# Autodesk Inventor assembly: A2017_T5_08
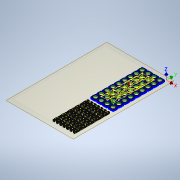
[picture p0: Inventor's stored thumbnail of the model, 180x180]
Saved by Autodesk Inventor 2022 (Build 260153000, 153)
## iProperties
Created: 2022-09-28
Part Number: A2017_T5_08
Document SubType Name: Assembly
Designer: Masato
Author: Masato
## Documents named in this file (6)
- C:\Users\ヨコオリク\Documents\CITBrains\SUSTAINA-OP\Cam\A2017_T5\A2017_T5_08.iam
- C:\Users\ヨコオリク\Documents\CITBrains\SUSTAINA-OP\Cam\DisposableBoard.ipt
- C:\Users\ヨコオリク\Documents\CITBrains\SUSTAINA-OP\LowerBody\Knee\Knee_clamp.ipt
- C:\Users\ヨコオリク\Documents\CITBrains\SUSTAINA-OP\UpperBody\Trunk\CrossRollerBearing\Inner_support_stand.ipt
- C:\Users\ヨコオリク\Documents\CITBrains\SUSTAINA-OP\UpperBody\Trunk\CrossRollerBearing\Outer_support_stand.ipt
- C:\Users\ヨコオリク\Documents\CITBrains\SUSTAINA-OP\LowerBody\Foot\Foot_root_block.ipt
## Components (103 placed, 5 different names)
1. DisposableBoard:1 — フラッシュ:1, フラッシュ:2, フラッシュ:3, フラッシュ:4, 正接:1, 正接:2, 正接:7, 正接:12, 正接:13, フラッシュ:5, フラッシュ:6, 正接:15, 正接:16
2. Inner_support_stand:1 — メイト:2, 挿入:1, 角度:2
3. Outer_support_stand:1 — メイト:1, 角度:1, 正接:1, 正接:2, 挿入:1
4. Inner_support_stand:2
5. Outer_support_stand:2
6. Inner_support_stand:3
7. Outer_support_stand:3
8. Inner_support_stand:4
9. Outer_support_stand:4
10. Inner_support_stand:5
11. Outer_support_stand:5
12. Inner_support_stand:6
13. Outer_support_stand:6
14. Inner_support_stand:7
15. Outer_support_stand:7
16. Inner_support_stand:8
17. Outer_support_stand:8
18. Inner_support_stand:9
19. Outer_support_stand:9
20. Inner_support_stand:10
21. Outer_support_stand:10
22. Knee_clamp:1 — メイト:4, メイト:5, メイト:6
23. Knee_clamp:2
24. Knee_clamp:3
25. Knee_clamp:4
26. Knee_clamp:38
27. Knee_clamp:21 — メイト:10, 正接:7, 正接:12, 正接:13
28. Knee_clamp:33
29. Knee_clamp:34
30. Knee_clamp:35
31. Knee_clamp:36
32. Knee_clamp:37
33. Foot_root_block:1 — メイト:11, フラッシュ:5, フラッシュ:6
34. Foot_root_block:2
35. Foot_root_block:3
36. Foot_root_block:4
37. Foot_root_block:5
38. Foot_root_block:6
39. Foot_root_block:7
40. Foot_root_block:8
41. Foot_root_block:9
42. Foot_root_block:10
43. Foot_root_block:11
44. Foot_root_block:12
45. Foot_root_block:13
46. Foot_root_block:14
47. Foot_root_block:15
48. Foot_root_block:16
49. Foot_root_block:17
50. Foot_root_block:18
51. Foot_root_block:19
52. Foot_root_block:20
53. Foot_root_block:21
54. Foot_root_block:22
55. Foot_root_block:23
56. Foot_root_block:24
57. Foot_root_block:25
58. Foot_root_block:26
59. Foot_root_block:27
60. Foot_root_block:28
61. Foot_root_block:29
62. Foot_root_block:30
63. Foot_root_block:31
64. Foot_root_block:32
65. Foot_root_block:33
66. Foot_root_block:34
67. Foot_root_block:35
68. Knee_clamp:39 — 角度:3, メイト:12, 正接:15
69. Knee_clamp:40
70. Knee_clamp:41
71. Knee_clamp:42
72. Knee_clamp:43
73. Knee_clamp:44
74. Knee_clamp:45
75. Knee_clamp:46
76. Knee_clamp:47
77. Knee_clamp:48
78. Knee_clamp:49
79. Knee_clamp:50
80. Knee_clamp:51
81. Knee_clamp:52
82. Knee_clamp:53
83. Knee_clamp:54
84. Knee_clamp:55
85. Knee_clamp:56
86. Knee_clamp:57
87. Knee_clamp:58
88. Knee_clamp:59
89. Knee_clamp:60
90. Knee_clamp:61
91. Knee_clamp:62
92. Knee_clamp:63
93. Knee_clamp:64
94. Knee_clamp:65
95. Knee_clamp:66
96. Knee_clamp:67
97. Knee_clamp:68
98. Knee_clamp:69
99. Knee_clamp:70
100. Knee_clamp:71 — 正接:16
101. Knee_clamp:72
102. Knee_clamp:73
103. Knee_clamp:74
## Component patterns: (10 elements, first: Inner_support_stand:1 + Outer_support_stand:1), (5 elements, first: Knee_clamp:1), (6 elements, first: Knee_clamp:21), (35 elements, first: Foot_root_block:1), (36 elements, first: Knee_clamp:39)
## Relationships (25: Mate 8, Tangent 7, Flush 6, Angle 3, Insert 1)
- フラッシュ:1 [Flush]: DisposableBoard:1
- フラッシュ:2 [Flush]: DisposableBoard:1
- フラッシュ:3 [Flush]: DisposableBoard:1
- フラッシュ:4 [Flush]: DisposableBoard:1
- メイト:1 [Mate]: Outer_support_stand:1
- メイト:2 [Mate]: Inner_support_stand:1
- メイト:4 [Mate]: Knee_clamp:1
- 角度:1 [Angle] (90 deg): Outer_support_stand:1
- 正接:1 [Tangent] (2 mm): DisposableBoard:1 ↔ Outer_support_stand:1
- 正接:2 [Tangent] (2 mm): DisposableBoard:1 ↔ Outer_support_stand:1
- 挿入:1 [Insert]: Inner_support_stand:1 ↔ Outer_support_stand:1
- 角度:2 [Angle] (0 deg): Inner_support_stand:1
- メイト:5 [Mate] (60.5 mm): Knee_clamp:1
- メイト:6 [Mate] (51.568 mm): Knee_clamp:1
- メイト:10 [Mate]: Knee_clamp:21
- 正接:7 [Tangent] (2 mm): DisposableBoard:1 ↔ Knee_clamp:21
- 正接:12 [Tangent] (2.1 mm): DisposableBoard:1 ↔ Knee_clamp:21
- 正接:13 [Tangent] (3 mm): DisposableBoard:1 ↔ Knee_clamp:21
- メイト:11 [Mate]: Foot_root_block:1
- フラッシュ:5 [Flush] (2 mm): DisposableBoard:1 ↔ Foot_root_block:1
- フラッシュ:6 [Flush] (2 mm): DisposableBoard:1 ↔ Foot_root_block:1
- 角度:3 [Angle] (45 deg): Knee_clamp:39
- メイト:12 [Mate]: Knee_clamp:39
- 正接:15 [Tangent] (2.5 mm): DisposableBoard:1 ↔ Knee_clamp:39
- 正接:16 [Tangent] (2.1 mm): DisposableBoard:1 ↔ Knee_clamp:71
